# Autodesk Inventor assembly: Mock Module PCB
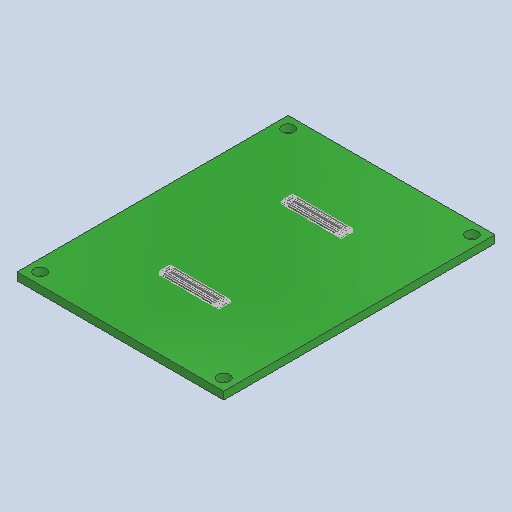
[picture p0: Inventor's stored thumbnail of the model, 512x512]
Saved by Autodesk Inventor 2022 (Build 260153000, 153)
## iProperties
Created: 2021-07-19
Part Number: Mock Module PCB
Document SubType Name: Assembly
Designer: Caleb
Author: Caleb
## Documents named in this file (3)
- C:\Users\Caleb\Desktop\nebraska-silicon-lab\Hardware\ETL\Module Assembly\Tamale Assembly Plate\Mock Module PCB.iam
- C:\Users\Caleb\Desktop\nebraska-silicon-lab\Hardware\ETL\Module Assembly\Tamale Assembly Plate\Mock Module PCB.ipt
- C:\Users\Caleb\Desktop\nebraska-silicon-lab\Hardware\ETL\ETL-SH-Design\3D-model\K3D-WP7B-S050VA1-V3_JAE_Proprietary v1_14.iam
## Components (3 placed, 2 different names)
1. Mock Module PCB:1 — Mate:1, Mate:2, Flush:1, Flush:2, Flush:3, Flush:4
2. K3D-WP7B-S050VA1-V3_JAE_Proprietary v1_14:1 [sub-assembly] — Mate:1, Flush:1, Flush:3
3. K3D-WP7B-S050VA1-V3_JAE_Proprietary v1_14:2 [sub-assembly] — Mate:2, Flush:2, Flush:4
## Relationships (6: Flush 4, Mate 2)
- Mate:1: Mock Module PCB:1 ↔ K3D-WP7B-S050VA1-V3_JAE_Proprietary v1_14:1
- Mate:2: Mock Module PCB:1 ↔ K3D-WP7B-S050VA1-V3_JAE_Proprietary v1_14:2
- Flush:1 (15.2019 mm): Mock Module PCB:1 ↔ K3D-WP7B-S050VA1-V3_JAE_Proprietary v1_14:1
- Flush:2 (15.2019 mm): Mock Module PCB:1 ↔ K3D-WP7B-S050VA1-V3_JAE_Proprietary v1_14:2
- Flush:3 (14.2 mm): Mock Module PCB:1 ↔ K3D-WP7B-S050VA1-V3_JAE_Proprietary v1_14:1
- Flush:4 (14.2 mm): Mock Module PCB:1 ↔ K3D-WP7B-S050VA1-V3_JAE_Proprietary v1_14:2
